# Autodesk Inventor assembly: Estante
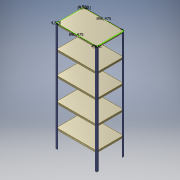
[picture p0: Inventor's stored thumbnail of the model, 180x180]
Saved by Autodesk Inventor 2016 (Build 200138000, 138)
## iProperties
Created: 2015-11-12
Part Number: Estante
Material: Genérico
Document SubType Name: Assembly
Designer: David
_SolveAssemblyDoc: Frame Generator Solve Assembly
_Version: 15.0.0
Author: David
## Documents named in this file (4)
- D:\mis documentos\david\computaciuon grafica\proyecto final\estantería\Estante.iam
- D:\mis documentos\david\computaciuon grafica\proyecto final\estantería\Esqueleto.ipt
- D:\mis documentos\david\computaciuon grafica\proyecto final\estantería\Estante\Frame\Frame0001.iam
- D:\mis documentos\david\computaciuon grafica\proyecto final\estantería\lámina.ipt
## Components (7 placed, 3 different names)
1. Esqueleto:1
2. Frame0001:1 [sub-assembly] — Nivelación:1
3. lámina:1 — Nivelación:1, Nivelación:2, Nivelación:3, Nivelación:4
4. lámina:2 — Nivelación:11, Nivelación:12, Nivelación:13
5. lámina:3 — Nivelación:5, Nivelación:6, Nivelación:7, Nivelación:8, Nivelación:9, Nivelación:10
6. lámina:4 — Nivelación:8, Nivelación:9, Nivelación:10, Nivelación:12, Nivelación:13
7. lámina:5 — Nivelación:2, Nivelación:3, Nivelación:4, Nivelación:5, Nivelación:6, Nivelación:7, Nivelación:11
## Relationships (13: Flush 13)
- Nivelación:1 [Flush]: Frame0001:1 ↔ lámina:1
- Nivelación:2 [Flush] (500 mm): lámina:1 ↔ lámina:5
- Nivelación:3 [Flush]: lámina:1 ↔ lámina:5
- Nivelación:4 [Flush]: lámina:1 ↔ lámina:5
- Nivelación:5 [Flush]: lámina:3 ↔ lámina:5
- Nivelación:6 [Flush] (500 mm): lámina:3 ↔ lámina:5
- Nivelación:7 [Flush]: lámina:3 ↔ lámina:5
- Nivelación:8 [Flush] (500 mm): lámina:3 ↔ lámina:4
- Nivelación:9 [Flush]: lámina:3 ↔ lámina:4
- Nivelación:10 [Flush]: lámina:3 ↔ lámina:4
- Nivelación:11 [Flush]: lámina:2 ↔ lámina:5
- Nivelación:12 [Flush] (500 mm): lámina:2 ↔ lámina:4
- Nivelación:13 [Flush]: lámina:2 ↔ lámina:4
